# Autodesk Inventor assembly: Drive Base
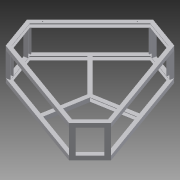
[picture p0: Inventor's stored thumbnail of the model, 180x180]
Saved by Autodesk Inventor 2013 (Build 170138000, 138)
## iProperties
Created: 2013-01-12
Part Number: Drive Base
Document SubType Name: Assembly
Designer: carneeki
Author: carneeki
## Documents named in this file (6)
- C:\Users\carneeki\Desktop\Kiwi Robot\Chassis\Chassis.iam
- C:\Users\carneeki\Desktop\Kiwi Robot\Chassis\Chassis Edge.ipt
- C:\Users\carneeki\Desktop\Kiwi Robot\Chassis\Chassis Corner.ipt
- C:\Users\carneeki\Desktop\Kiwi Robot\Chassis\Chassis Vertical Support.ipt
- C:\Users\carneeki\Desktop\Kiwi Robot\Chassis\Chassis Cross Support.ipt
- C:\Users\carneeki\Desktop\Kiwi Robot\Chassis\Chassis Rear Edge.ipt
## Components (21 placed, 21 different names)
1. Chassis Cross Support:A — Mate:228, Mate:229, Flush:17, Mate:230, Mate:231, Mate:232, Mate:235
2. Chassis Corner - Short:A - Upper — Mate:213, Mate:214, Mate:215, Flush:15, Mate:224, Mate:225
3. Chassis Corner - Short:A - Lower — Mate:187, Flush:4, Mate:193, Mate:194, Flush:5, Mate:195, Mate:196, Mate:200, Mate:201, Flush:8, Flush:9, Mate:208
4. Chassis Edge:A - Upper — Flush:14, Mate:222, Mate:223
5. Chassis Edge:A - Lower — Flush:3, Mate:191, Mate:192, Mate:197, Flush:6, Mate:211, Mate:235
6. Chassis Vertical:A - Left — Mate:201, Flush:9, Mate:209, Mate:214
7. Chassis Vertical:A - Right — Mate:200, Flush:8, Mate:208, Mate:213, Mate:215
8. Chassis Cross Support:B — Mate:232, Mate:233, Flush:18
9. Chassis Corner:B - Lower — Mate:189, Mate:190, Flush:2, Flush:3, Mate:191, Mate:192, Mate:202, Mate:203, Flush:12, Flush:13, Mate:207, Mate:212
10. Chassis Corner:B - Upper — Mate:216, Mate:217, Mate:218, Flush:16, Mate:226, Mate:227
11. Chassis Edge:B - Lower — Flush:4, Mate:193, Mate:194, Mate:198, Flush:7, Mate:209, Mate:210
12. Chassis Edge:B - Upper — Flush:15, Mate:224, Mate:225
13. Chassis Vertical:B - Left — Mate:202, Flush:12, Mate:206, Mate:216, Mate:217
14. Chassis Vertical:B - Right — Mate:203, Flush:13, Mate:207, Mate:212, Mate:218
15. Chassis Cross Support:C — Mate:228, Mate:229, Flush:17, Mate:230, Mate:231, Mate:233, Flush:18, Mate:234
16. Chassis Corner:C - Lower — Mate:197, Flush:6, Mate:198, Flush:7, Mate:204, Mate:205, Flush:10, Flush:11
17. Chassis Corner:C - Upper — Mate:219, Mate:220, Mate:221, Flush:14, Mate:222, Mate:223
18. Chassis Edge:C - Upper — Flush:16, Mate:226, Mate:227
19. Chassis Edge:C - Lower — Mate:187, Mate:189, Mate:190, Flush:2, Flush:5, Mate:195, Mate:196, Mate:206, Mate:234
20. Chassis Vertical:C - Left — Mate:204, Flush:11, Mate:211, Mate:221
21. Chassis Vertical:C - Right — Mate:205, Flush:10, Mate:210, Mate:219, Mate:220
## Relationships (64: Mate 47, Flush 17)
- Mate:187: Chassis Corner - Short:A - Lower ↔ Chassis Edge:C - Lower
- Mate:189: Chassis Corner:B - Lower ↔ Chassis Edge:C - Lower
- Mate:190: Chassis Corner:B - Lower ↔ Chassis Edge:C - Lower
- Flush:2: Chassis Corner:B - Lower ↔ Chassis Edge:C - Lower
- Flush:3: Chassis Edge:A - Lower ↔ Chassis Corner:B - Lower
- Mate:191: Chassis Edge:A - Lower ↔ Chassis Corner:B - Lower
- Mate:192: Chassis Edge:A - Lower ↔ Chassis Corner:B - Lower
- Flush:4: Chassis Corner - Short:A - Lower ↔ Chassis Edge:B - Lower
- Mate:193: Chassis Corner - Short:A - Lower ↔ Chassis Edge:B - Lower
- Mate:194: Chassis Corner - Short:A - Lower ↔ Chassis Edge:B - Lower
- Flush:5: Chassis Corner - Short:A - Lower ↔ Chassis Edge:C - Lower
- Mate:195: Chassis Corner - Short:A - Lower ↔ Chassis Edge:C - Lower
- Mate:196: Chassis Corner - Short:A - Lower ↔ Chassis Edge:C - Lower
- Mate:197: Chassis Edge:A - Lower ↔ Chassis Corner:C - Lower
- Flush:6: Chassis Edge:A - Lower ↔ Chassis Corner:C - Lower
- Mate:198: Chassis Edge:B - Lower ↔ Chassis Corner:C - Lower
- Flush:7: Chassis Edge:B - Lower ↔ Chassis Corner:C - Lower
- Mate:200: Chassis Corner - Short:A - Lower ↔ Chassis Vertical:A - Right
- Mate:201: Chassis Corner - Short:A - Lower ↔ Chassis Vertical:A - Left
- Mate:202: Chassis Corner:B - Lower ↔ Chassis Vertical:B - Left
- Mate:203: Chassis Corner:B - Lower ↔ Chassis Vertical:B - Right
- Mate:204: Chassis Corner:C - Lower ↔ Chassis Vertical:C - Left
- Mate:205: Chassis Corner:C - Lower ↔ Chassis Vertical:C - Right
- Flush:8: Chassis Corner - Short:A - Lower ↔ Chassis Vertical:A - Right
- Flush:9: Chassis Corner - Short:A - Lower ↔ Chassis Vertical:A - Left
- Flush:10: Chassis Corner:C - Lower ↔ Chassis Vertical:C - Right
- Flush:11: Chassis Corner:C - Lower ↔ Chassis Vertical:C - Left
- Flush:12: Chassis Corner:B - Lower ↔ Chassis Vertical:B - Left
- Flush:13: Chassis Corner:B - Lower ↔ Chassis Vertical:B - Right
- Mate:206: Chassis Vertical:B - Left ↔ Chassis Edge:C - Lower
- Mate:207: Chassis Corner:B - Lower ↔ Chassis Vertical:B - Right
- Mate:208: Chassis Corner - Short:A - Lower ↔ Chassis Vertical:A - Right
- Mate:209: Chassis Vertical:A - Left ↔ Chassis Edge:B - Lower
- Mate:210: Chassis Edge:B - Lower ↔ Chassis Vertical:C - Right
- Mate:211: Chassis Edge:A - Lower ↔ Chassis Vertical:C - Left
- Mate:212: Chassis Corner:B - Lower ↔ Chassis Vertical:B - Right
- Mate:213: Chassis Corner - Short:A - Upper ↔ Chassis Vertical:A - Right
- Mate:214: Chassis Corner - Short:A - Upper ↔ Chassis Vertical:A - Left
- Mate:215: Chassis Corner - Short:A - Upper ↔ Chassis Vertical:A - Right
- Mate:216: Chassis Corner:B - Upper ↔ Chassis Vertical:B - Left
- Mate:217: Chassis Corner:B - Upper ↔ Chassis Vertical:B - Left
- Mate:218: Chassis Corner:B - Upper ↔ Chassis Vertical:B - Right
- Mate:219: Chassis Corner:C - Upper ↔ Chassis Vertical:C - Right
- Mate:220: Chassis Corner:C - Upper ↔ Chassis Vertical:C - Right
- Mate:221: Chassis Corner:C - Upper ↔ Chassis Vertical:C - Left
- Flush:14: Chassis Edge:A - Upper ↔ Chassis Corner:C - Upper
- Mate:222: Chassis Edge:A - Upper ↔ Chassis Corner:C - Upper
- Mate:223: Chassis Edge:A - Upper ↔ Chassis Corner:C - Upper
- Flush:15: Chassis Corner - Short:A - Upper ↔ Chassis Edge:B - Upper
- Mate:224: Chassis Corner - Short:A - Upper ↔ Chassis Edge:B - Upper
- Mate:225: Chassis Corner - Short:A - Upper ↔ Chassis Edge:B - Upper
- Flush:16: Chassis Corner:B - Upper ↔ Chassis Edge:C - Upper
- Mate:226: Chassis Corner:B - Upper ↔ Chassis Edge:C - Upper
- Mate:227: Chassis Corner:B - Upper ↔ Chassis Edge:C - Upper
- Mate:228: Chassis Cross Support:A ↔ Chassis Cross Support:C
- Mate:229: Chassis Cross Support:A ↔ Chassis Cross Support:C
- Flush:17: Chassis Cross Support:A ↔ Chassis Cross Support:C
- Mate:230: Chassis Cross Support:A ↔ Chassis Cross Support:C
- Mate:231: Chassis Cross Support:A ↔ Chassis Cross Support:C
- Mate:232: Chassis Cross Support:A ↔ Chassis Cross Support:B
- Mate:233: Chassis Cross Support:B ↔ Chassis Cross Support:C
- Flush:18: Chassis Cross Support:B ↔ Chassis Cross Support:C
- Mate:234: Chassis Cross Support:C ↔ Chassis Edge:C - Lower
- Mate:235: Chassis Cross Support:A ↔ Chassis Edge:A - Lower
